# Autodesk Inventor assembly: V4.0-trebuchet-printable
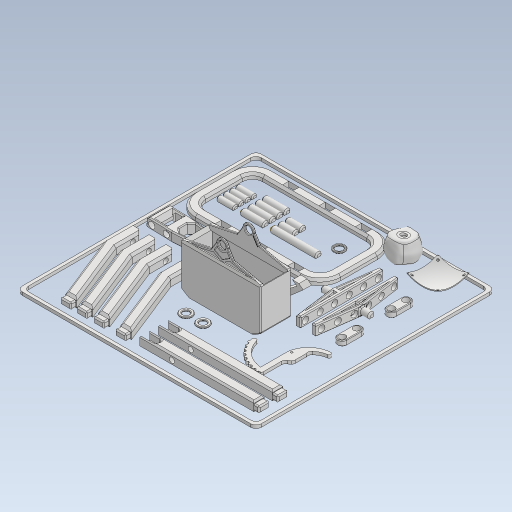
[picture p0: Inventor's stored thumbnail of the model, 512x512]
Saved by Autodesk Inventor 2023 (Build 270158030, 158C)
## iProperties
Created: 2024-12-20
Part Number: V4.0-trebuchet-printable
Document SubType Name: Assembly
Designer: Imogen Heard
Author: Imogen Heard
## Documents named in this file (21)
- C:\Users\dheard\Documents\0004-inventor\3D-CAD-main\trebuchet\V4.0-trebuchet-printable.iam
- C:\Users\dheard\Documents\0004-inventor\3D-CAD-main\trebuchet\pins.ipt
- C:\Users\dheard\Documents\0004-inventor\3D-CAD-main\trebuchet\bolder.ipt
- C:\Users\dheard\Documents\0004-inventor\3D-CAD-main\trebuchet\sling.ipt
- C:\Users\dheard\Documents\0004-inventor\3D-CAD-main\unicorn-horn\washers.ipt
- C:\Users\dheard\Documents\0004-inventor\3D-CAD-main\trebuchet\V2-baseplate.ipt
- C:\Users\dheard\Documents\0004-inventor\3D-CAD-main\trebuchet\V2-upright-a.ipt
- C:\Users\dheard\Documents\0004-inventor\3D-CAD-main\trebuchet\V2-a-frame.ipt
- C:\Users\dheard\Documents\0004-inventor\3D-CAD-main\trebuchet\V2-pivot-a.ipt
- C:\Users\dheard\Documents\0004-inventor\3D-CAD-main\trebuchet\V2-throw-arm.ipt
- C:\Users\dheard\Documents\0004-inventor\3D-CAD-main\trebuchet\v2-ratchet.ipt
- C:\Users\dheard\Documents\0004-inventor\3D-CAD-main\trebuchet\V2-counterweight.ipt
- C:\Users\dheard\Documents\0004-inventor\3D-CAD-main\trebuchet\V2-pivot-mirror.ipt
- C:\Users\dheard\Documents\0004-inventor\3D-CAD-main\trebuchet\V2-upright-mirror.ipt
- C:\Users\dheard\Documents\0004-inventor\3D-CAD-main\trebuchet\V2-a-frame-B.ipt
- C:\Users\dheard\Documents\0004-inventor\3D-CAD-main\trebuchet\V2-a-frame-C.ipt
- C:\Users\dheard\Documents\0004-inventor\3D-CAD-main\trebuchet\V2-a-frame-D.ipt
- C:\Users\dheard\Documents\0004-inventor\3D-CAD-main\trebuchet\V2-spacer-A.ipt
- C:\Users\dheard\Documents\0004-inventor\3D-CAD-main\trebuchet\V2-spacer-B.ipt
- C:\Users\dheard\Documents\0004-inventor\3D-CAD-main\trebuchet\throw-ring.ipt
- C:\Users\dheard\Documents\0004-inventor\3D-CAD-main\trebuchet\border.ipt
## Components (21 placed, 20 different names)
1. pins:1 — Flush:7, Flush:25, Flush:26, Flush:27, Flush:28, Flush:29, Flush:30, Flush:31, Flush:32, Flush:33, Flush:34, Flush:35, Flush:36, Flush:37, Flush:38, Flush:39
2. bolder:1
3. sling:1
4. washers:1 — Flush:19
5. V2-baseplate:1 — Flush:1
6. V2-upright-a:1 — Flush:15, Flush:17
7. V2-a-frame:1 — Flush:11, Flush:12, Flush:14
8. V2-pivot-a:1 — Flush:5, Mate:4
9. V2-throw-arm:1 — Flush:4
10. v2-ratchet:1 — Flush:3, Flush:5, Angle:1, Flush:24
11. V2-counterweight:1 — Flush:2
12. V2-pivot-mirror:1 — Flush:6, Mate:3, Mate:4, Mate:5
13. V2-upright-mirror:1 — Flush:16, Flush:17, Mate:1
14. V2-a-frame-B:1 — Flush:13, Flush:14
15. V2-a-frame-C:1 — Flush:8, Flush:10
16. V2-a-frame-D:1 — Flush:9, Flush:10, Flush:11, Flush:12
17. V2-spacer-A:1 — Flush:20, Mate:5, Flush:23
18. V2-spacer-B:1 — Flush:22, Flush:23
19. washers:2 — Flush:21
20. throw-ring:1 — Flush:18
21. border:1 — Flush:1, Flush:2, Flush:3, Flush:4, Flush:6, Flush:7, Flush:8, Flush:9, Flush:13, Flush:15, Flush:16, Mate:1, Flush:18, Flush:19, Flush:20, Flush:21, Flush:22, Mate:3, Angle:1, Flush:24, Flush:25, Flush:26, Flush:27, Flush:28, Flush:29, Flush:30, Flush:31, Flush:32, Flush:33, Flush:34, Flush:35, Flush:36, Flush:37, Flush:38, Flush:39
## Relationships (44: Flush 39, Mate 4, Angle 1)
- Flush:1: V2-baseplate:1 ↔ border:1
- Flush:2: V2-counterweight:1 ↔ border:1
- Flush:3: v2-ratchet:1 ↔ border:1
- Flush:4: V2-throw-arm:1 ↔ border:1
- Flush:5: V2-pivot-a:1 ↔ v2-ratchet:1
- Flush:6: V2-pivot-mirror:1 ↔ border:1
- Flush:7: pins:1 ↔ border:1
- Flush:8: V2-a-frame-C:1 ↔ border:1
- Flush:9: V2-a-frame-D:1 ↔ border:1
- Flush:10: V2-a-frame-C:1 ↔ V2-a-frame-D:1
- Flush:11: V2-a-frame:1 ↔ V2-a-frame-D:1
- Flush:12: V2-a-frame:1 ↔ V2-a-frame-D:1
- Flush:13: V2-a-frame-B:1 ↔ border:1
- Flush:14: V2-a-frame:1 ↔ V2-a-frame-B:1
- Flush:15: V2-upright-a:1 ↔ border:1
- Flush:16: V2-upright-mirror:1 ↔ border:1
- Flush:17: V2-upright-a:1 ↔ V2-upright-mirror:1
- Mate:1 (7 mm): V2-upright-mirror:1 ↔ border:1
- Flush:18: throw-ring:1 ↔ border:1
- Flush:19: washers:1 ↔ border:1
- Flush:20: V2-spacer-A:1 ↔ border:1
- Flush:21: washers:2 ↔ border:1
- Flush:22: V2-spacer-B:1 ↔ border:1
- Mate:3 (60 mm): V2-pivot-mirror:1 ↔ border:1
- Mate:4 (10 mm): V2-pivot-a:1 ↔ V2-pivot-mirror:1
- Mate:5 (27 mm): V2-pivot-mirror:1 ↔ V2-spacer-A:1
- Flush:23: V2-spacer-A:1 ↔ V2-spacer-B:1
- Angle:1 (0 deg): v2-ratchet:1 ↔ border:1
- Flush:24: v2-ratchet:1 ↔ border:1
- Flush:25: pins:1 ↔ border:1
- Flush:26: pins:1 ↔ border:1
- Flush:27: pins:1 ↔ border:1
- Flush:28: pins:1 ↔ border:1
- Flush:29: pins:1 ↔ border:1
- Flush:30: pins:1 ↔ border:1
- Flush:31: pins:1 ↔ border:1
- Flush:32: pins:1 ↔ border:1
- Flush:33: pins:1 ↔ border:1
- Flush:34: pins:1 ↔ border:1
- Flush:35: pins:1 ↔ border:1
- Flush:36: pins:1 ↔ border:1
- Flush:37: pins:1 ↔ border:1
- Flush:38: pins:1 ↔ border:1
- Flush:39: pins:1 ↔ border:1
